# Autodesk Inventor assembly: outsideHand
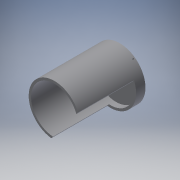
[picture p0: Inventor's stored thumbnail of the model, 180x180]
Saved by Autodesk Inventor 2016 (Build 200138000, 138)
## iProperties
Created: 2016-11-10
Part Number: outsideHand
Material: 一般
Document SubType Name: Assembly
Designer: Daisuke
Author: Daisuke
## Documents named in this file (5)
- C:\Users\Daisuke\Documents\GitHub\CAD\Hand\ver1\outsideHand.iam
- C:\Users\Daisuke\Documents\GitHub\CAD\Hand\ver1\outsideBottom.ipt
- C:\Users\Daisuke\Documents\GitHub\CAD\Hand\ver1\outsideCover.ipt
- C:\Users\Daisuke\Documents\GitHub\CAD\Hand\ver1\UFL08 -Housing.ipt
- C:\Users\Daisuke\Documents\GitHub\CAD\Hand\ver1\Servo.iam
## Components (4 placed, 4 different names)
1. outsideBottom:1 — 挿入:1, 挿入:2, 挿入:3, 挿入:6, 挿入:7, 挿入:8, 挿入:9, メイト:1
2. outsideCover:1 — 挿入:1, メイト:1
3. UFL08 -Housing:1 — 挿入:2, 挿入:3
4. Servo:1 [sub-assembly] — 挿入:6, 挿入:7, 挿入:8, 挿入:9
## Relationships (8: Insert 7, Mate 1)
- 挿入:1 [Insert]: outsideBottom:1 ↔ outsideCover:1
- 挿入:2 [Insert]: outsideBottom:1 ↔ UFL08 -Housing:1
- 挿入:3 [Insert]: outsideBottom:1 ↔ UFL08 -Housing:1
- 挿入:6 [Insert]: outsideBottom:1 ↔ Servo:1
- 挿入:7 [Insert]: outsideBottom:1 ↔ Servo:1
- 挿入:8 [Insert]: outsideBottom:1 ↔ Servo:1
- 挿入:9 [Insert]: outsideBottom:1 ↔ Servo:1
- メイト:1 [Mate]: outsideBottom:1 ↔ outsideCover:1
